# Autodesk Inventor assembly: Indicator Assembly
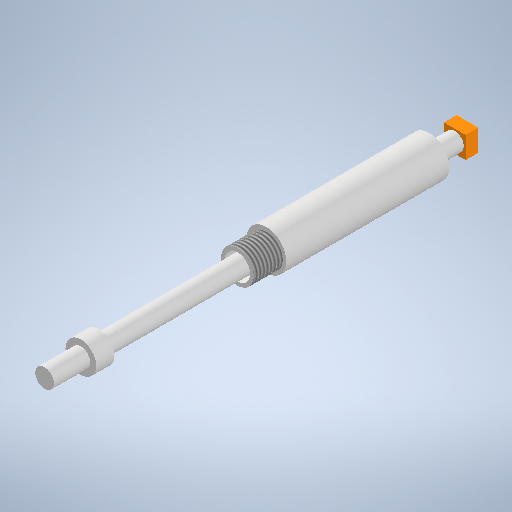
[picture p0: Inventor's stored thumbnail of the model, 512x512]
Saved by Autodesk Inventor 2025.2 (Build 292293000, 293)
## iProperties
Created: 2025-04-06
Part Number: Indicator Assembly
Document SubType Name: Assembly
Designer: eason
Author: eason
## Documents named in this file (5)
- C:\Users\eason\Desktop\Code\Unojoy-Simulator-Rig\CAD\Indicator\Indicator Assembly.iam
- C:\Users\eason\Desktop\Code\Unojoy-Simulator-Rig\CAD\Indicator\Button.ipt
- C:\Users\eason\Desktop\Code\Unojoy-Simulator-Rig\CAD\Indicator\Hat.ipt
- C:\Users\eason\Desktop\Code\Unojoy-Simulator-Rig\CAD\Indicator\Rod.ipt
- C:\Users\eason\Desktop\Code\Unojoy-Simulator-Rig\CAD\Indicator\Stalk.ipt
## Components (4 placed, 4 different names)
1. Button:1 — Insert:1, Mate:1, Mate:2, Flush:1, Flush:2
2. Hat:1 — Insert:1, Cylindrical:1
3. Rod:1 — Cylindrical:1, Cylindrical:2
4. Stalk:1 — Cylindrical:2, Flush:2
## Relationships (7: Mate 2, Flush 2, CylindricalJoint 2, Insert 1)
- Insert:1: Button:1 ↔ Hat:1
- Mate:1: Button:1
- Mate:2: Button:1
- Flush:1: Button:1
- Cylindrical:1: Hat:1 ↔ Rod:1
- Cylindrical:2: Rod:1 ↔ Stalk:1
- Flush:2 (-60 mm): Button:1 ↔ Stalk:1
